# Autodesk Inventor assembly: 1x10
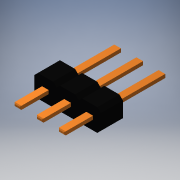
[picture p0: Inventor's stored thumbnail of the model, 180x180]
Saved by Autodesk Inventor 2016 (Build 200138000, 138)
## iProperties
Created: 2014-07-19
Part Number: 1x10
Document SubType Name: Assembly
Designer: Sawaiz Syed
Author: Sawaiz Syed
## Documents named in this file (2)
- C:\Users\Jonathan\Documents\Projects\nonmodular\coincidenceCounter\cad\electronics\2.54 breakaway\1x10.iam
- C:\Users\Jonathan\Documents\Projects\nonmodular\coincidenceCounter\cad\electronics\2.54 breakaway\1x1.iam
## Components (3 placed, 1 different names)
1. 1x1:1 [sub-assembly]
2. 1x1:2 [sub-assembly]
3. 1x1:3 [sub-assembly]
## Component patterns: (3 elements, first: 1x1:1)
